# Autodesk Inventor assembly: Aufhängung_Version2
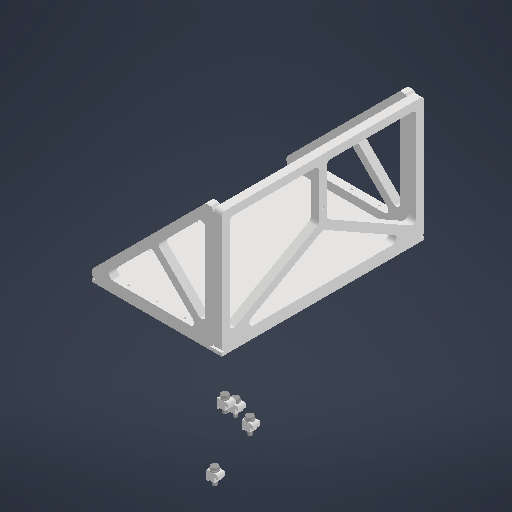
[picture p0: Inventor's stored thumbnail of the model, 512x512]
Saved by Autodesk Inventor 2027 (Build 310192060, 192F)
## iProperties
Created: 2026-07-21
Part Number: Aufhängung_Version2
Document SubType Name: Assembly
Designer: kw
Author: kw
## Documents named in this file (5)
- C:\Users\kw\OneDrive\Documents\Uni\Masterthesis\Spezialisierungsmodul\InventorZeichnungen\Koppeltest_Halterung\Aufhängung_Version2.iam
- C:\Users\kw\OneDrive\Documents\Uni\Masterthesis\Spezialisierungsmodul\InventorZeichnungen\Koppeltest_Halterung\Aufhängung.ipt
- C:\Users\kw\OneDrive\Documents\Uni\Masterthesis\Spezialisierungsmodul\InventorZeichnungen\Koppeltest_Halterung\Aufhängung_Gerüst.ipt
- C:\Users\kw\OneDrive\Documents\Uni\Masterthesis\Spezialisierungsmodul\InventorZeichnungen\Koppeltest_Halterung\TeflonPlate.ipt
- C:\Users\kw\OneDrive\Documents\Uni\Masterthesis\Spezialisierungsmodul\InventorZeichnungen\Koppeltest_Halterung\Pratze_ISO-K160\Pratze_ISO-K160.ipt
## Components (8 placed, 4 different names)
1. Aufhängung:1 — Mate:3, Flush:5, Flush:6
2. Aufhängung_Gerüst:1 — Mate:1, Flush:1, Flush:2
3. TeflonPlate:1 — Mate:1, Flush:1, Flush:2, Mate:2, Flush:3, Flush:4, Mate:3, Flush:5, Flush:6
4. Aufhängung_Gerüst:2 — Mate:2, Flush:3, Flush:4
5. Pratze_ISO-K160:1
6. Pratze_ISO-K160:2
7. Pratze_ISO-K160:3
8. Pratze_ISO-K160:4
## Relationships (9: Flush 6, Mate 3)
- Mate:1: Aufhängung_Gerüst:1 ↔ TeflonPlate:1
- Flush:1: Aufhängung_Gerüst:1 ↔ TeflonPlate:1
- Flush:2 (20 mm): Aufhängung_Gerüst:1 ↔ TeflonPlate:1
- Mate:2: TeflonPlate:1 ↔ Aufhängung_Gerüst:2
- Flush:3: TeflonPlate:1 ↔ Aufhängung_Gerüst:2
- Flush:4 (20 mm): TeflonPlate:1 ↔ Aufhängung_Gerüst:2
- Mate:3: Aufhängung:1 ↔ TeflonPlate:1
- Flush:5: Aufhängung:1 ↔ TeflonPlate:1
- Flush:6: Aufhängung:1 ↔ TeflonPlate:1
